# Autodesk Inventor assembly: Red Scale
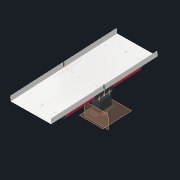
[picture p0: Inventor's stored thumbnail of the model, 180x180]
Saved by Autodesk Inventor 2021 (Build 250183000, 183)
## iProperties
Created: 2021-05-23
Part Number: Red Scale
Document SubType Name: Assembly
Designer: max
Author: max
Revision Number: ANY
## Documents named in this file (13)
- C:\Users\max\Desktop\Vex\TiP FieldCAD\Scales\Red Scale.iam
- C:\Users\max\Desktop\Vex\Library 1.2\Structure\Hardware\Screw Steel - Star\Screw 8-32 Steel .375.ipt
- C:\Users\max\Desktop\Vex\Library 1.2\Structure\Hardware\Screw Steel - Star.ipt
- C:\Users\max\Desktop\Vex\Library 1.2\Structure\Hardware\Screw Steel - Star\Screw 8-32 Steel 1.000.ipt
- C:\Users\max\Desktop\Vex\Library 1.2\Structure\Standoff\Standoff .75.ipt
- C:\Users\max\Desktop\Vex\Library 1.2\Structure\Standoff.ipt
- C:\Users\max\Desktop\Vex\TiP FieldCAD\Scales\Field Tile Mounting Plate.ipt
- C:\Users\max\Desktop\Vex\TiP FieldCAD\Scales\Scale Base.iam
- C:\Users\max\Desktop\Vex\TiP FieldCAD\Scales\Scale Pivot Linkage.ipt
- C:\Users\max\Desktop\Vex\TiP FieldCAD\Scales\Scale Pivot Coupler.ipt
- C:\Users\max\Desktop\Vex\Library 1.2\Structure\Standoff\Standoff 1.5.ipt
- C:\Users\max\Desktop\Vex\TiP FieldCAD\Scales\Scale Platform.iam
- C:\Users\max\Desktop\Vex\TiP FieldCAD\Scales\Perimeter Mounting Bracket.ipt
## Components (29 placed, 10 different names)
1. Screw 8-32 Steel .375:1 — Insert:1
2. Screw 8-32 Steel 1.000:2 — Mate:4, Mate:5, Mate:6, Mate:7
3. Standoff .75:1 — Insert:2, Mate:4, Mate:8
4. Field Tile Mounting Plate:1 — Insert:1, Insert:2
5. Scale Base:1 [sub-assembly] — Mate:5, Mate:6, Mate:7, Mate:8, Mate:13, Mate:14, Mate:15, Mate:16, Mate:20, Flush:9, Flush:10, Mate:39
6. Scale Pivot Linkage:1 — Mate:11, Mate:12, Mate:42
7. Scale Pivot Coupler:1 — Mate:9, Mate:10, Mate:11, Mate:12, Insert:3, Insert:4, Mate:18, Mate:19, Mate:20, Tangent:1, Flush:7, Flush:12, Mate:39, Mate:41, Flush:13
8. Standoff 1.5:2 — Mate:9, Mate:10
9. Screw 8-32 Steel .375:3 — Insert:3
10. Screw 8-32 Steel .375:4 — Insert:4
11. Screw 8-32 Steel .375:5 — Mate:16, Flush:3, Mate:18
12. Screw 8-32 Steel .375:6 — Mate:15, Flush:2, Flush:3, Mate:19, Tangent:1
13. Screw 8-32 Steel .375:7 — Mate:14, Flush:1
14. Screw 8-32 Steel .375:8 — Mate:13, Flush:1, Flush:2
15. Scale Platform:1 [sub-assembly] — Mate:40, Mate:41, Mate:42, Flush:13
16. Screw 8-32 Steel 1.000:10
17. Scale Base:2 [sub-assembly] — Insert:9, Insert:10, Flush:9, Flush:10
18. Scale Pivot Coupler:2 — Mate:37, Mate:38, Flush:7, Flush:12, Mate:40
19. Standoff 1.5:4
20. Screw 8-32 Steel .375:11
21. Screw 8-32 Steel .375:12
22. Screw 8-32 Steel .375:13
23. Screw 8-32 Steel .375:14
24. Screw 8-32 Steel .375:15
25. Screw 8-32 Steel .375:16
26. Perimeter Mounting Bracket:1 — Insert:11, Mate:36
27. Standoff 1.5:5 — Insert:9, Insert:11
28. Standoff 1.5:6 — Insert:10, Mate:36
29. Scale Pivot Linkage:2 — Mate:37, Mate:38
## Relationships (57: Mate 35, Flush 11, Insert 9, Tangent 2)
- Insert:1: Screw 8-32 Steel .375:1 ↔ Field Tile Mounting Plate:1
- Insert:2: Standoff .75:1 ↔ Field Tile Mounting Plate:1
- Mate:4: Screw 8-32 Steel 1.000:2 ↔ Standoff .75:1
- Mate:5: Screw 8-32 Steel 1.000:2 ↔ Scale Base:1
- Mate:6: Screw 8-32 Steel 1.000:2 ↔ Scale Base:1
- Mate:7: Screw 8-32 Steel 1.000:2 ↔ Scale Base:1
- Mate:8: Standoff .75:1 ↔ Scale Base:1
- Mate:9: Scale Pivot Coupler:1 ↔ Standoff 1.5:2
- Mate:10: Scale Pivot Coupler:1 ↔ Standoff 1.5:2
- Mate:11: Scale Pivot Linkage:1 ↔ Scale Pivot Coupler:1
- Mate:12: Scale Pivot Linkage:1 ↔ Scale Pivot Coupler:1
- Insert:3: Scale Pivot Coupler:1 ↔ Screw 8-32 Steel .375:3
- Insert:4: Scale Pivot Coupler:1 ↔ Screw 8-32 Steel .375:4
- Mate:13: Scale Base:1 ↔ Screw 8-32 Steel .375:8
- Mate:14: Scale Base:1 ↔ Screw 8-32 Steel .375:7
- Mate:15: Scale Base:1 ↔ Screw 8-32 Steel .375:6
- Mate:16: Scale Base:1 ↔ Screw 8-32 Steel .375:5
- Flush:1: Screw 8-32 Steel .375:7 ↔ Screw 8-32 Steel .375:8
- Flush:2: Screw 8-32 Steel .375:6 ↔ Screw 8-32 Steel .375:8
- Flush:3: Screw 8-32 Steel .375:5 ↔ Screw 8-32 Steel .375:6
- Mate:18: Scale Pivot Coupler:1 ↔ Screw 8-32 Steel .375:5
- Mate:19: Scale Pivot Coupler:1 ↔ Screw 8-32 Steel .375:6
- Mate:20: Scale Base:1 ↔ Scale Pivot Coupler:1
- Tangent:1: Scale Pivot Coupler:1 ↔ Screw 8-32 Steel .375:6
- [Mate]: Screw 8-32 Steel 1.000:10 ↔ Scale Base:2
- [Mate]: Screw 8-32 Steel 1.000:10 ↔ Scale Base:2
- [Mate]: Screw 8-32 Steel 1.000:10 ↔ Scale Base:2
- [Mate]: Scale Pivot Coupler:2 ↔ Standoff 1.5:4
- [Mate]: Scale Pivot Coupler:2 ↔ Standoff 1.5:4
- [Insert]: Scale Pivot Coupler:2 ↔ Screw 8-32 Steel .375:11
- [Insert]: Scale Pivot Coupler:2 ↔ Screw 8-32 Steel .375:12
- [Mate]: Scale Base:2 ↔ Screw 8-32 Steel .375:16
- [Mate]: Scale Base:2 ↔ Screw 8-32 Steel .375:15
- [Mate]: Scale Base:2 ↔ Screw 8-32 Steel .375:14
- [Mate]: Scale Base:2 ↔ Screw 8-32 Steel .375:13
- [Flush]: Screw 8-32 Steel .375:15 ↔ Screw 8-32 Steel .375:16
- [Flush]: Screw 8-32 Steel .375:14 ↔ Screw 8-32 Steel .375:16
- [Flush]: Screw 8-32 Steel .375:13 ↔ Screw 8-32 Steel .375:14
- [Mate]: Scale Pivot Coupler:2 ↔ Screw 8-32 Steel .375:13
- [Mate]: Scale Pivot Coupler:2 ↔ Screw 8-32 Steel .375:14
- [Mate]: Scale Base:2 ↔ Scale Pivot Coupler:2
- [Tangent]: Scale Pivot Coupler:2 ↔ Screw 8-32 Steel .375:14
- Insert:9: Scale Base:2 ↔ Standoff 1.5:5
- Insert:10: Scale Base:2 ↔ Standoff 1.5:6
- Insert:11: Perimeter Mounting Bracket:1 ↔ Standoff 1.5:5
- Mate:36: Perimeter Mounting Bracket:1 ↔ Standoff 1.5:6
- Mate:37: Scale Pivot Coupler:2 ↔ Scale Pivot Linkage:2
- Mate:38: Scale Pivot Coupler:2 ↔ Scale Pivot Linkage:2
- Flush:7: Scale Pivot Coupler:1 ↔ Scale Pivot Coupler:2
- Flush:9: Scale Base:1 ↔ Scale Base:2
- Flush:10: Scale Base:1 ↔ Scale Base:2
- Flush:12: Scale Pivot Coupler:1 ↔ Scale Pivot Coupler:2
- Mate:39 (-1.778 mm): Scale Base:1 ↔ Scale Pivot Coupler:1
- Mate:40: Scale Platform:1 ↔ Scale Pivot Coupler:2
- Mate:41: Scale Pivot Coupler:1 ↔ Scale Platform:1
- Mate:42: Scale Pivot Linkage:1 ↔ Scale Platform:1
- Flush:13: Scale Pivot Coupler:1 ↔ Scale Platform:1
## Named parameters: d121_d28 = 0 mm, d122_d16 = 0 mm, d123_d17 = 0 mm, d124_d18 = 0 mm, d125_d19 = 0 mm, d126_d20 = 0 mm, d127_d21 = 0 mm, d128_d22 = 0 mm, d129_d23 = 0 mm, d131_d25 = 0 mm, d132_d26 = 0 mm, d133_d27 = 0 mm, d134_d15 = 0 mm, d135_d7 = 0 mm, d136_d8 = 0 mm, d137_d9 = 0 mm, d139_d11 = 0 mm, d140_d12 = 0 mm
